# Autodesk Inventor assembly: Idler Gear Assembly
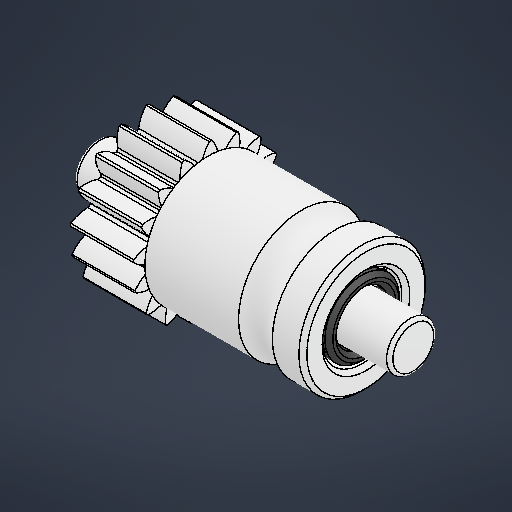
[picture p0: Inventor's stored thumbnail of the model, 512x512]
Saved by Autodesk Inventor 2026 (Build 300175050, 175E)
## iProperties
Created: 2025-05-09
Part Number: Idler Gear Assembly
Document SubType Name: Assembly
Designer: AdminForWorker
Title: Idler Gear Assembly
Author: AdminForWorker
## Documents named in this file (4)
- C:\Users\Joshua Eah\Documents\GitHub\Voron-0\CAD\Master Assembly\Toolhead\Subassemblies\Idler Gear Assembly.iam
- C:\Users\Joshua Eah\Documents\GitHub\Voron-0\CAD\Master Assembly\Toolhead\Parts\Extruder\Idler Gear Shaft.ipt
- C:\Users\Joshua Eah\Documents\GitHub\Voron-0\CAD\Master Assembly\Toolhead\Parts\Extruder\Needle Bearing.ipt
- C:\Users\Joshua Eah\Documents\GitHub\Voron-0\CAD\Master Assembly\Toolhead\Parts\Extruder\Idler Gear.ipt
## Components (4 placed, 3 different names)
1. Idler Gear Shaft:1 — Mate:1
2. Needle Bearing:1 — Insert:1, Insert:2
3. Needle Bearing:2 — Insert:1
4. Idler Gear:1 — Mate:1, Insert:2
## Relationships (3: Insert 2, Mate 1)
- Insert:1: Needle Bearing:1 ↔ Needle Bearing:2
- Mate:1: Idler Gear Shaft:1 ↔ Idler Gear:1
- Insert:2: Needle Bearing:1 ↔ Idler Gear:1
